# Autodesk Inventor assembly: chamber
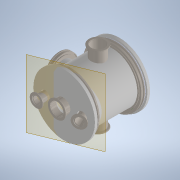
[picture p0: Inventor's stored thumbnail of the model, 180x180]
Saved by Autodesk Inventor 2021 (Build 250183000, 183)
## iProperties
Created: 2024-02-21
Part Number: chamber
Document SubType Name: Assembly
Designer: Sebastián
Author: Sebastián
## Documents named in this file (8)
- C:\Users\Sebastián\Documents\Inventor\PLD SAP\chamber.iam
- C:\Users\Sebastián\Documents\Inventor\PLD SAP\chamber.ipt
- C:\Users\Sebastián\Documents\Inventor\PLD_Chamber\Hositrad_ISO-K160-154.ipt
- C:\Users\Sebastián\Documents\Inventor\PLD SAP\KF40-40_mandri.ipt
- C:\Users\Sebastián\Documents\Inventor\PLD SAP\ISO63.iam
- C:\Users\Sebastián\Documents\Inventor\PLD SAP\Hositrad_ISO160AV.ipt
- C:\Users\Sebastián\Documents\Inventor\PLD SAP\top_flange.iam
- C:\Users\Sebastián\Documents\Inventor\PLD SAP\bottom_cover.iam
## Components (9 placed, 7 different names)
1. chamber:1 — Rotational:1, Rotational:2, Cylindrical:1, Cylindrical:2, Mate:1, Mate:2, Cylindrical:3, Mate:3
2. Hositrad_ISO-K160-154:1 — Rotational:1, Rotational:4, Rotational:6
3. Hositrad_ISO-K160-154:2 — Rotational:2, Rotational:5
4. KF40-40_mandri:1 — Cylindrical:1, Mate:2
5. KF40-40_mandri:2 — Cylindrical:2, Mate:1
6. ISO63:1 [sub-assembly] — Cylindrical:3, Mate:3
7. Hositrad_ISO160AV:2 — Rotational:4
8. top_flange:1 [sub-assembly] — Rotational:5
9. bottom_cover:1 [sub-assembly] — Rotational:6
## Relationships (11: RevoluteJoint 5, CylindricalJoint 3, Mate 3)
- Rotational:1 [RevoluteJoint]: chamber:1 ↔ Hositrad_ISO-K160-154:1
- Rotational:2 [RevoluteJoint]: chamber:1 ↔ Hositrad_ISO-K160-154:2
- Cylindrical:1: chamber:1 ↔ KF40-40_mandri:1
- Cylindrical:2: chamber:1 ↔ KF40-40_mandri:2
- Mate:1 (2 mm): chamber:1 ↔ KF40-40_mandri:2
- Mate:2 (-2 mm): chamber:1 ↔ KF40-40_mandri:1
- Cylindrical:3: chamber:1 ↔ ISO63:1
- Mate:3: chamber:1 ↔ ISO63:1
- Rotational:4 [RevoluteJoint]: Hositrad_ISO-K160-154:1 ↔ Hositrad_ISO160AV:2
- Rotational:5 [RevoluteJoint]: Hositrad_ISO-K160-154:2 ↔ top_flange:1
- Rotational:6 [RevoluteJoint]: Hositrad_ISO-K160-154:1 ↔ bottom_cover:1
